# Autodesk Inventor assembly: s-assy-guide_plates
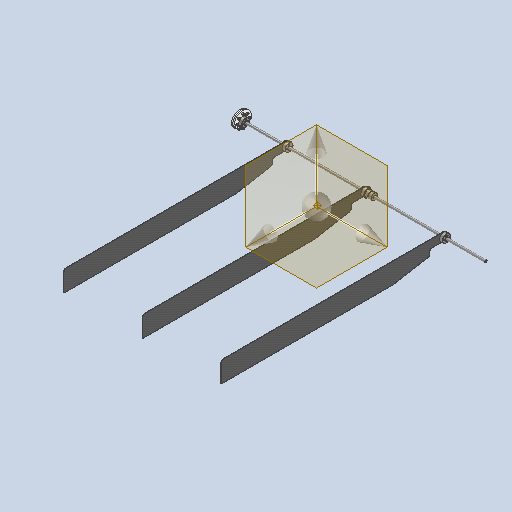
[picture p0: Inventor's stored thumbnail of the model, 512x512]
Saved by Autodesk Inventor 2022 (Build 260153000, 153)
## iProperties
Created: 2021-10-03
Part Number: s-assy-guide_plates
Document SubType Name: Assembly
Designer: Yuta Kage
Mass: 361.904 g
Surface Area: 1916.34 cm^2
Volume: 114.455 cm^3
Density: 3.16197 g/cm^3
Author: Yuta Kage
## Documents named in this file (6)
- C:\Users\yuta0\Documents\GitHub\catchrobo_hardware\assy-shooter\s-assy-guide_plates.iam
- C:\Users\yuta0\Documents\GitHub\catchrobo_hardware\assy-shooter\s-assy-guide.iam
- C:\Users\yuta0\Documents\GitHub\catchrobo_hardware\assy-shooter\CPRC16-6-6.iam
- C:\Users\yuta0\Documents\GitHub\catchrobo_hardware\assy-shooter\s-assy-guide_coupling.iam
- C:\Users\yuta0\Documents\GitHub\catchrobo_hardware\assy-shooter\SFR6-321.ipt
- C:\Users\yuta0\Documents\GitHub\catchrobo_hardware\assy-shooter\SFR6-285_s.ipt
## Components (7 placed, 5 different names)
1. CPRC16-6-6:1 [sub-assembly] — メイト:3, 角度:1, メイト:8
2. s-assy-guide_coupling:1 [sub-assembly] — フラッシュ:2, フラッシュ:3, メイト:4
3. SFR6-285_s:1
4. SFR6-321:1 — メイト:4, メイト:5, メイト:8
5. s-assy-guide:1 [sub-assembly] — フラッシュ:3, メイト:5
6. s-assy-guide:2 [sub-assembly] — メイト:3
7. s-assy-guide:3 [sub-assembly]
## Component patterns: (3 elements, first: s-assy-guide:1)
## Relationships (9: Mate 6, Flush 2, Angle 1)
- メイト:3 [Mate]: CPRC16-6-6:1 ↔ s-assy-guide:2
- 角度:1 [Angle] (0 deg): CPRC16-6-6:1
- フラッシュ:2 [Flush]: s-assy-guide_coupling:1
- フラッシュ:3 [Flush] (-112.8 mm): s-assy-guide_coupling:1 ↔ s-assy-guide:1
- メイト:4 [Mate]: s-assy-guide_coupling:1 ↔ SFR6-321:1
- メイト:5 [Mate]: SFR6-321:1 ↔ s-assy-guide:1
- [Mate]: SFR6-285_s:1 ↔ s-assy-guide:2
- [Mate]: SFR6-285_s:1 ↔ SFR6-321:1
- メイト:8 [Mate] (-8 mm): CPRC16-6-6:1 ↔ SFR6-321:1
